# Autodesk Inventor assembly: Heat sink assembly
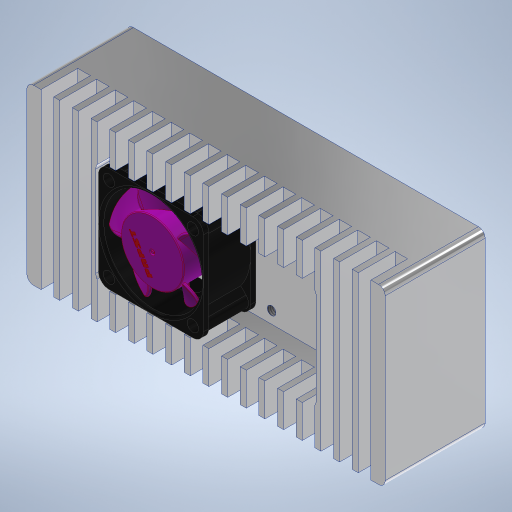
[picture p0: Inventor's stored thumbnail of the model, 512x512]
Saved by Autodesk Inventor 2023.4 (Build 274418000, 418)
## iProperties
Created: 2025-01-07
Part Number: Heat sink assembly
Document SubType Name: Assembly
Designer: mavericks
Author: mavericks
## Documents named in this file (3)
- C:\Users\jmcintyr\Desktop\2025-ReefScape---CAD\Heat Sink\Heat sink assembly.iam
- C:\Users\jmcintyr\Desktop\2025-ReefScape---CAD\Heat Sink\Heat sink.ipt
- C:\Users\jmcintyr\Desktop\2025-ReefScape---CAD\Heat Sink\12V fan 40mm_sq.ipt
## Components (2 placed, 2 different names)
1. Heat sink:1 — Insert:1, Insert:2
2. 12V fan 40mm_sq:2 — Insert:1, Insert:2
## Relationships (2: Insert 2)
- Insert:1: Heat sink:1 ↔ 12V fan 40mm_sq:2
- Insert:2: Heat sink:1 ↔ 12V fan 40mm_sq:2
